# Autodesk Inventor assembly: dribl-2-2
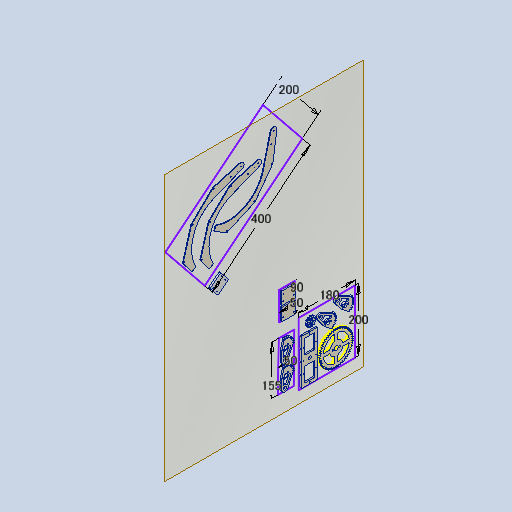
[picture p0: Inventor's stored thumbnail of the model, 512x512]
Saved by Autodesk Inventor 2025.2 (Build 292293000, 293)
## iProperties
Created: 2025-05-15
Part Number: dribl-2-2
Document SubType Name: Assembly
Designer: haruy
Author: haruy
## Documents named in this file (8)
- C:\Users\haruy\Documents\ロボコン\NHK2025\cad\cnc\dribl-2-2.iam
- C:\Users\haruy\Documents\ロボコン\NHK2025\cad\nagahisa\hand\grab\hand-grab-v5-Plate-1.ipt
- C:\Users\haruy\Documents\ロボコン\NHK2025\cad\nagahisa\hand\grab\000-hand-grab-v5\デザイン アクセラレータ\平歯車1.iam
- C:\Users\haruy\Documents\ロボコン\NHK2025\cad\nagahisa\dribl\000-dribl-v2\デザイン アクセラレータ\平歯車13.ipt
- C:\Users\haruy\Documents\ロボコン\NHK2025\cad\nagahisa\dribl\000-dribl-v2\デザイン アクセラレータ\平歯車23.ipt
- C:\Users\haruy\Documents\ロボコン\NHK2025\cad\nagahisa\dribl\dribl-v4-Plate-3.ipt
- C:\Users\haruy\Documents\ロボコン\NHK2025\cad\nagahisa\hand\grab\hand-grab-v5-Plate-4.ipt
- C:\Users\haruy\Documents\ロボコン\NHK2025\cad\nagahisa\hand\grab\000-hand-grab-v5\デザイン アクセラレータ\平歯車11.ipt
## Components (13 placed, 6 different names)
1. hand-grab-v5-Plate-1:1 — フラッシュ:1, フラッシュ:2, フラッシュ:6
2. 平歯車:1 [sub-assembly] — フラッシュ:2, フラッシュ:3, フラッシュ:4
3. 平歯車:2 [sub-assembly] — フラッシュ:3
4. 平歯車1:1 — フラッシュ:4, フラッシュ:5
5. 平歯車2:1 — フラッシュ:5
6. dribl-v4-Plate-3:1 — フラッシュ:6, フラッシュ:7, フラッシュ:8, メイト:1
7. dribl-v4-Plate-3:2 — フラッシュ:7, フラッシュ:8, メイト:1, フラッシュ:14, フラッシュ:15
8. hand-grab-v5-Plate-4:1 — フラッシュ:9, フラッシュ:10, 角度:1, フラッシュ:12
9. hand-grab-v5-Plate-4:2 — フラッシュ:10, 角度:1, フラッシュ:11, 角度:2, フラッシュ:13
10. hand-grab-v5-Plate-4:3 — フラッシュ:11, 角度:2
11. dribl-v4-Plate-3:3 — フラッシュ:12, フラッシュ:13
12. 平歯車1:2 — フラッシュ:14, フラッシュ:15, フラッシュ:16, フラッシュ:17
13. 平歯車1:3 — フラッシュ:16, フラッシュ:17
## Relationships (20: Flush 17, Angle 2, Mate 1)
- フラッシュ:1 [Flush]: hand-grab-v5-Plate-1:1
- フラッシュ:2 [Flush]: hand-grab-v5-Plate-1:1 ↔ 平歯車:1
- フラッシュ:3 [Flush]: 平歯車:1 ↔ 平歯車:2
- フラッシュ:4 [Flush]: 平歯車:1 ↔ 平歯車1:1
- フラッシュ:5 [Flush]: 平歯車1:1 ↔ 平歯車2:1
- フラッシュ:6 [Flush]: hand-grab-v5-Plate-1:1 ↔ dribl-v4-Plate-3:1
- フラッシュ:7 [Flush]: dribl-v4-Plate-3:1 ↔ dribl-v4-Plate-3:2
- フラッシュ:8 [Flush]: dribl-v4-Plate-3:1 ↔ dribl-v4-Plate-3:2
- メイト:1 [Mate] (5 mm): dribl-v4-Plate-3:1 ↔ dribl-v4-Plate-3:2
- フラッシュ:9 [Flush]: hand-grab-v5-Plate-4:1
- フラッシュ:10 [Flush]: hand-grab-v5-Plate-4:1 ↔ hand-grab-v5-Plate-4:2
- 角度:1 [Angle] (0 deg): hand-grab-v5-Plate-4:1 ↔ hand-grab-v5-Plate-4:2
- フラッシュ:11 [Flush]: hand-grab-v5-Plate-4:2 ↔ hand-grab-v5-Plate-4:3
- 角度:2 [Angle] (130 deg): hand-grab-v5-Plate-4:2 ↔ hand-grab-v5-Plate-4:3
- フラッシュ:12 [Flush]: hand-grab-v5-Plate-4:1 ↔ dribl-v4-Plate-3:3
- フラッシュ:13 [Flush]: hand-grab-v5-Plate-4:2 ↔ dribl-v4-Plate-3:3
- フラッシュ:14 [Flush]: dribl-v4-Plate-3:2 ↔ 平歯車1:2
- フラッシュ:15 [Flush]: dribl-v4-Plate-3:2 ↔ 平歯車1:2
- フラッシュ:16 [Flush]: 平歯車1:2 ↔ 平歯車1:3
- フラッシュ:17 [Flush]: 平歯車1:2 ↔ 平歯車1:3
